# Autodesk Inventor assembly: CONVEYOR-01
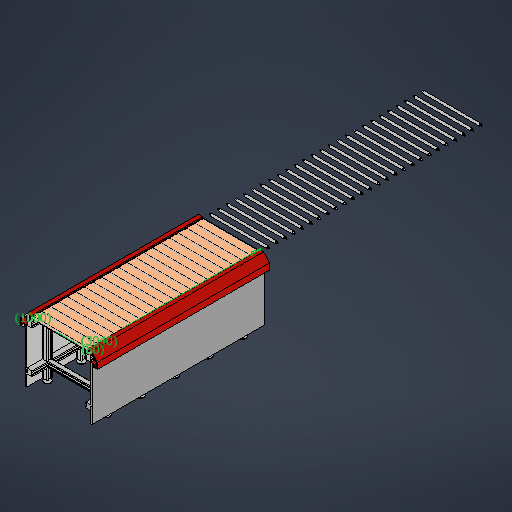
[picture p0: Inventor's stored thumbnail of the model, 512x512]
Saved by Autodesk Inventor 2025 (Build 290162000, 162)
## iProperties
RuleStatus: InUse
Created: 2024-05-06
Part Number: CONVEYOR-01
Document SubType Name: Assembly
Designer: zulet
AfterComponentReplace0: Rebuild
Author: zulet
rollerSeparation: 80,000 mm
conveyorLength: 3040,000 mm
rollerLength: 1000,000 mm
## Documents named in this file (8)
- D:\UNAL\2024-1S\APM\Digital Factory\Conveyor System\CONVEYOR\CONVEYOR-1000x3040x1140.iam
- D:\UNAL\2024-1S\APM\Digital Factory\Conveyor System\CONVEYOR STRUCTURE.ipt
- D:\UNAL\2024-1S\APM\Digital Factory\Conveyor System\CONVEYOR ROLLER.ipt
- D:\UNAL\2024-1S\APM\Digital Factory\Conveyor System\CONVEYOR SURFACE.ipt
- D:\UNAL\2024-1S\APM\Digital Factory\Conveyor System\CONVEYOR.iam
- D:\UNAL\2024-1S\APM\Digital Factory\Conveyor System\CONVEYOR STRUCTURE\CONVEYOR STRUCTURE-01.ipt
- D:\UNAL\2024-1S\APM\Digital Factory\Conveyor System\CONVEYOR ROLLER\CR-1000.ipt
- D:\UNAL\2024-1S\APM\Digital Factory\Conveyor System\CONVEYOR SURFACE\CONVEYOR SURFACE-1000x3040.ipt
## Components (49 placed, 3 different names)
1. CONVEYOR STRUCTURE-01:1 — Mate:1, Mate:2, Rigid:1
2. CONVEYOR SURFACE-1000x3040:1 — Rigid:1
3. CR-1000:1 — Mate:1, Mate:2
4. CR-1000:2
5. CR-1000:3
6. CR-1000:4
7. CR-1000:5
8. CR-1000:6
9. CR-1000:7
10. CR-1000:8
11. CR-1000:9
12. CR-1000:10
13. CR-1000:11
14. CR-1000:12
15. CR-1000:13
16. CR-1000:14
17. CR-1000:15
18. CR-1000:16
19. CR-1000:17
20. CR-1000:18
21. CR-1000:19
22. CR-1000:20
23. CR-1000:21
24. CR-1000:22
25. CR-1000:23
26. CR-1000:24
27. CR-1000:25
28. CR-1000:26
29. CR-1000:27
30. CR-1000:28
31. CR-1000:29
32. CR-1000:30
33. CR-1000:31
34. CR-1000:32
35. CR-1000:33
36. CR-1000:34
37. CR-1000:35
38. CR-1000:36
39. CR-1000:37
40. CR-1000:38
41. CR-1000:40
42. CR-1000:41
43. CR-1000:42
44. CR-1000:43
45. CR-1000:44
46. CR-1000:45
47. CR-1000:46
48. CR-1000:47
49. CR-1000:48
## Component patterns: (47 elements, first: CR-1000:1)
## Relationships (3: Mate 2, WeldJoint 1)
- Mate:1: CONVEYOR STRUCTURE-01:1 ↔ CR-1000:1
- Mate:2: CONVEYOR STRUCTURE-01:1 ↔ CR-1000:1
- Rigid:1 [WeldJoint]: CONVEYOR STRUCTURE-01:1 ↔ CONVEYOR SURFACE-1000x3040:1
